# Autodesk Inventor assembly: Bumper Assembly2 (24x28 robot)
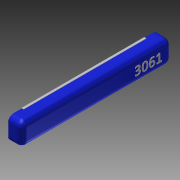
[picture p0: Inventor's stored thumbnail of the model, 180x180]
Saved by Autodesk Inventor 2013 (Build 170138000, 138)
## iProperties
Created: 2013-01-06
Part Number: Bumper Assembly2 (24x28 robot)
Document SubType Name: Assembly
Designer: Moses
Mass: 1284.45 g
Surface Area: 11568.4 cm^2
Volume: 5857.21 cm^3
Density: 0.219293 g/cm^3
Author: Moses
## Documents named in this file (5)
- C:\Users\Moses\Documents\GitHub\frc2013CAD\Robot Chassis and Drivetrain\Chassis\Bumpers\Bumper Assembly2 (24x28 robot).iam
- C:\Users\Moses\Documents\GitHub\frc2013CAD\Robot Chassis and Drivetrain\Chassis\Bumpers\Bumper Wood Backing Part2 (24x28 robot).ipt
- C:\Users\Moses\Documents\GitHub\frc2013CAD\Robot Chassis and Drivetrain\Chassis\Bumpers\Pool Noodle Part2 (24x28 robot).ipt
- C:\Users\Moses\Documents\GitHub\frc2013CAD\Robot Chassis and Drivetrain\Chassis\Bumpers\Bumper Metal Edge Part2 (24x28 robot).ipt
- C:\Users\Moses\Documents\GitHub\frc2013CAD\Robot Chassis and Drivetrain\Chassis\Bumpers\Bumper Cover Part2 (24x28 robot).ipt
## Components (6 placed, 4 different names)
1. Bumper Wood Backing Part2 (24x28 robot):1 — Mate:1, Mate:2, Tangent:1, Tangent:2, Tangent:4, Mate:1, Mate:2
2. Pool Noodle Part2 (24x28 robot):1 — Mate:1, Tangent:1, Tangent:3, Tangent:4, Tangent:5
3. Pool Noodle Part2 (24x28 robot):2 — Mate:2, Tangent:2, Tangent:3
4. Bumper Cover Part2 (24x28 robot):1 — Mate:1, Mate:2, Tangent:5, Mate:3, Mate:4, Mate:5, Mate:6, Mate:7
5. Bumper Metal Edge Part2 (24x28 robot):1 — Mate:5, Mate:6, Flush:1
6. Bumper Metal Edge Part2 (24x28 robot):2 — Mate:3, Mate:4, Flush:1, Mate:7
## Relationships (15: Mate 9, Tangent 5, Flush 1)
- Mate:1 (-9.525 mm): Bumper Wood Backing Part2 (24x28 robot):1 ↔ Pool Noodle Part2 (24x28 robot):1
- Mate:2 (-9.525 mm): Bumper Wood Backing Part2 (24x28 robot):1 ↔ Pool Noodle Part2 (24x28 robot):2
- Tangent:1: Bumper Wood Backing Part2 (24x28 robot):1 ↔ Pool Noodle Part2 (24x28 robot):1
- Tangent:2: Bumper Wood Backing Part2 (24x28 robot):1 ↔ Pool Noodle Part2 (24x28 robot):2
- Tangent:3: Pool Noodle Part2 (24x28 robot):1 ↔ Pool Noodle Part2 (24x28 robot):2
- Tangent:4: Bumper Wood Backing Part2 (24x28 robot):1 ↔ Pool Noodle Part2 (24x28 robot):1
- Mate:1: Bumper Wood Backing Part2 (24x28 robot):1 ↔ Bumper Cover Part2 (24x28 robot):1
- Mate:2: Bumper Wood Backing Part2 (24x28 robot):1 ↔ Bumper Cover Part2 (24x28 robot):1
- Tangent:5: Pool Noodle Part2 (24x28 robot):1 ↔ Bumper Cover Part2 (24x28 robot):1
- Mate:3: Bumper Cover Part2 (24x28 robot):1 ↔ Bumper Metal Edge Part2 (24x28 robot):2
- Mate:4: Bumper Cover Part2 (24x28 robot):1 ↔ Bumper Metal Edge Part2 (24x28 robot):2
- Mate:5: Bumper Cover Part2 (24x28 robot):1 ↔ Bumper Metal Edge Part2 (24x28 robot):1
- Mate:6: Bumper Cover Part2 (24x28 robot):1 ↔ Bumper Metal Edge Part2 (24x28 robot):1
- Flush:1: Bumper Metal Edge Part2 (24x28 robot):1 ↔ Bumper Metal Edge Part2 (24x28 robot):2
- Mate:7 (46.0375 mm): Bumper Cover Part2 (24x28 robot):1 ↔ Bumper Metal Edge Part2 (24x28 robot):2
